# Autodesk Inventor assembly: arms assembly for plow
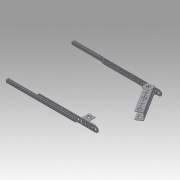
[picture p0: Inventor's stored thumbnail of the model, 180x180]
Saved by Autodesk Inventor 2016 (Build 200138000, 138)
## iProperties
Created: 2015-10-24
Part Number: arms assembly for plow
Document SubType Name: Assembly
Designer: Delta
Author: Delta
## Documents named in this file (5)
- C:\Robotics\CAD\2015-16\custom cad parts\arms assembly for plow.iam
- C:\Robotics\CAD\2015-16\COTSParts\Tetrix\Pitsco Education-739271.iam
- C:\Robotics\CAD\2015-16\COTSParts\Actobotics\585 parts\585398.ipt
- C:\Robotics\CAD\2015-16\COTSParts\Tetrix\User Library-TX 160 MM Channel.ipt
- C:\Robotics\CAD\2015-16\COTSParts\Tetrix\Tetrix channel 32mm.ipt
## Components (7 placed, 4 different names)
1. Pitsco Education-739271:2 [sub-assembly] — Mate:2, Insert:3, Insert:6
2. Pitsco Education-739271:3 [sub-assembly] — Insert:1, Insert:7
3. 585398:1 — Mate:2
4. 585398:2
5. User Library-TX 160 MM Channel:1 — Insert:8
6. Tetrix channel 32mm:1 — Insert:1, Insert:7
7. Tetrix channel 32mm:3 — Insert:3, Insert:6, Insert:8
## Relationships (6: Insert 5, Mate 1)
- Mate:2: Pitsco Education-739271:2 ↔ 585398:1
- Insert:1: Pitsco Education-739271:3 ↔ Tetrix channel 32mm:1
- Insert:3: Pitsco Education-739271:2 ↔ Tetrix channel 32mm:3
- Insert:6: Pitsco Education-739271:2 ↔ Tetrix channel 32mm:3
- Insert:7: Pitsco Education-739271:3 ↔ Tetrix channel 32mm:1
- Insert:8: User Library-TX 160 MM Channel:1 ↔ Tetrix channel 32mm:3
